# Autodesk Inventor assembly: Robot_Rev2
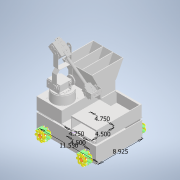
[picture p0: Inventor's stored thumbnail of the model, 180x180]
Saved by Autodesk Inventor 2020 (Build 240168000, 168)
## iProperties
Created: 2021-12-14
Part Number: Robot_Rev2
Document SubType Name: Assembly
Designer: danie
Author: danie
## Documents named in this file (9)
- C:\Users\danie\Documents\Capstone\Solidworks\Robot_Rev2.iam
- C:\Users\danie\Documents\Capstone\Solidworks\Lower Chassis_2.ipt
- C:\Users\danie\Documents\Capstone\Solidworks\UpperChassis_Base_2.ipt
- C:\Users\danie\Documents\Capstone\Solidworks\ShootingMech_Housing3.ipt
- C:\Users\danie\Documents\Capstone\Solidworks\BeadCompartments_3.ipt
- C:\Users\danie\Documents\Capstone\Solidworks\False_Bottom_2.ipt
- C:\Users\danie\Documents\Capstone\Solidworks\AL5D_2017_12_17.iam
- C:\Users\danie\Documents\Capstone\Solidworks\MECHANUM WHEEL.iam
- C:\Users\danie\Documents\Capstone\Solidworks\TurntableandBase.iam
## Components (11 placed, 8 different names)
1. Lower Chassis_2:1 — Rigid:1
2. UpperChassis_Base_2:1 — Rigid:1, Rigid:2
3. ShootingMech_Housing3:1 — Rigid:2
4. BeadCompartments_3:1
5. False_Bottom_2:1
6. AL5D_2017_12_17:1 [sub-assembly]
7. MECHANUM WHEEL:1 [sub-assembly]
8. MECHANUM WHEEL:2 [sub-assembly]
9. MECHANUM WHEEL:3 [sub-assembly]
10. MECHANUM WHEEL:4 [sub-assembly]
11. TurntableandBase:1 [sub-assembly]
## Relationships (2: WeldJoint 2)
- Rigid:1 [WeldJoint] (9.144 mm): Lower Chassis_2:1 ↔ UpperChassis_Base_2:1
- Rigid:2 [WeldJoint]: UpperChassis_Base_2:1 ↔ ShootingMech_Housing3:1
